# Autodesk Inventor assembly: waterjet assembly version
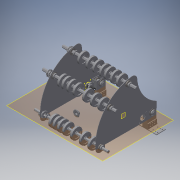
[picture p0: Inventor's stored thumbnail of the model, 180x180]
Saved by Autodesk Inventor 2018 (Build 220112000, 112)
## iProperties
Created: 2020-01-24
Part Number: waterjet assembly version
Document SubType Name: Assembly
Designer: s-2513225
Author: s-2513225
## Documents named in this file (11)
- \\studenthome\students\S-2513225\GitHub\2020CAD\Over bumper intake\Assembly\waterjet assembly version.iam
- \\studenthome\students\S-2513225\GitHub\2020CAD\Over bumper intake\Parts\waterjet wall.ipt
- \\studenthome\students\S-2513225\GitHub\2020CAD\Over bumper intake\Parts\0_500_Hex_ID_x_1_125_OD_x_0_313_WD_Flanged_Bearing_v2_217-3875.ipt
- \\studenthome\students\S-2513225\GitHub\2020CAD\Over bumper intake\Parts\hex shaft 1.ipt
- \\studenthome\students\S-2513225\GitHub\2020CAD\Over bumper intake\Parts\banebots 400 - 2 3-8 replacement.ipt
- \\studenthome\students\S-2513225\GitHub\2020CAD\Over bumper intake\Parts\anchor point.ipt
- \\studenthome\students\S-2513225\GitHub\2020CAD\Over bumper intake\Parts\hex 2.ipt
- \\studenthome\students\S-2513225\GitHub\2020CAD\Over bumper intake\Parts\2in bracket.ipt
- \\studenthome\students\S-2513225\GitHub\2020CAD\Over bumper intake\Parts\VersaPlanetary_v2_Single_Stage_10_1_with_775_Series.iam
- \\studenthome\students\S-2513225\GitHub\2020CAD\Over bumper intake\Parts\_16t_Aluminum_Hub_Sprocket_25_Chain_1_2_Hex_Bore_217-2642.ipt
- \\studenthome\students\S-2513225\GitHub\2020CAD\Over bumper intake\Parts\Clamping_Shaft_Collar_-_1_2_Hex_ID_217-2737.ipt
## Components (67 placed, 10 different names)
1. waterjet wall:1 — Mate:2, Mate:4, Mate:5, Mate:6, Mate:7, Mate:8, Mate:9, Mate:26, Mate:90, Mate:91, Mate:97, Mate:108, Mate:109, Flush:11, Flush:12, Mate:154, Mate:157, Mate:165
2. waterjet wall:2 — Mate:17, Mate:18, Mate:19, Mate:20, Mate:21, Mate:22, Mate:26, Mate:88, Mate:89, Mate:99, Flush:13, Mate:166
3. 0_500_Hex_ID_x_1_125_OD_x_0_313_WD_Flanged_Bearing_v2_217-3875:1 — Mate:5, Mate:7, Mate:10, Mate:15, Mate:150
4. 0_500_Hex_ID_x_1_125_OD_x_0_313_WD_Flanged_Bearing_v2_217-3875:2 — Mate:6, Mate:9, Mate:12, Mate:14, Mate:152
5. 0_500_Hex_ID_x_1_125_OD_x_0_313_WD_Flanged_Bearing_v2_217-3875:3 — Mate:4, Mate:8, Mate:11, Mate:13
6. 0_500_Hex_ID_x_1_125_OD_x_0_313_WD_Flanged_Bearing_v2_217-3875:4 — Mate:19, Mate:21, Mate:24
7. 0_500_Hex_ID_x_1_125_OD_x_0_313_WD_Flanged_Bearing_v2_217-3875:5 — Mate:18, Mate:20, Mate:23, Mate:25
8. 0_500_Hex_ID_x_1_125_OD_x_0_313_WD_Flanged_Bearing_v2_217-3875:6 — Mate:17, Mate:22
9. hex shaft 1:1 — Mate:12, Mate:14, Mate:23, Mate:25, Mate:37, Mate:53, Mate:68, Mate:72, Mate:73, Mate:74, Mate:75, Mate:76, Mate:77, Mate:78, Mate:104, Mate:105, Mate:106, Mate:107, Flush:11, Mate:122, Mate:123, Mate:138, Mate:139, Mate:153, Mate:161
10. hex shaft 1:2 — Mate:10, Mate:15, Mate:27, Mate:28, Mate:29, Mate:30, Mate:39, Mate:42, Mate:43, Mate:44, Mate:45, Mate:46, Mate:61, Mate:62, Mate:63, Mate:64, Mate:132, Mate:133, Mate:134, Mate:135, Mate:136, Mate:147, Mate:151, Mate:162
11. hex shaft 1:3 — Mate:11, Mate:13, Mate:24, Mate:31, Mate:32, Mate:33, Mate:34, Mate:40, Mate:47, Mate:48, Mate:49, Mate:50, Mate:51, Mate:65, Mate:66, Mate:69, Mate:70, Mate:124, Mate:125, Mate:126, Mate:127, Mate:128, Mate:129, Mate:137, Mate:148, Mate:163
12. banebots 400 - 2 3-8 replacement:1 — Mate:27, Mate:42
13. banebots 400 - 2 3-8 replacement:2 — Mate:30, Mate:43
14. banebots 400 - 2 3-8 replacement:3 — Mate:31, Mate:50
15. banebots 400 - 2 3-8 replacement:4 — Mate:29, Mate:44
16. banebots 400 - 2 3-8 replacement:5 — Mate:40, Mate:51
17. banebots 400 - 2 3-8 replacement:6 — Mate:28, Mate:46
18. banebots 400 - 2 3-8 replacement:7 — Mate:34, Mate:47
19. banebots 400 - 2 3-8 replacement:8 — Mate:32, Mate:48
20. banebots 400 - 2 3-8 replacement:9 — Mate:39, Mate:45
21. banebots 400 - 2 3-8 replacement:10 — Mate:73, Mate:78
22. banebots 400 - 2 3-8 replacement:11 — Mate:37, Mate:53
23. banebots 400 - 2 3-8 replacement:12 — Mate:75, Mate:76
24. banebots 400 - 2 3-8 replacement:13 — Mate:105, Mate:106
25. banebots 400 - 2 3-8 replacement:14 — Mate:33, Mate:49
26. banebots 400 - 2 3-8 replacement:15 — Mate:104, Mate:107
27. banebots 400 - 2 3-8 replacement:16 — Mate:61, Mate:63
28. banebots 400 - 2 3-8 replacement:17 — Mate:62, Mate:64
29. banebots 400 - 2 3-8 replacement:18 — Mate:66, Mate:70
30. banebots 400 - 2 3-8 replacement:19 — Mate:65, Mate:69
31. banebots 400 - 2 3-8 replacement:20 — Mate:74, Mate:77
32. banebots 400 - 2 3-8 replacement:21 — Mate:68, Mate:72
33. anchor point:1 — Mate:80, Mate:81, Mate:97, Flush:5, Mate:101, Flush:6, Flush:9, Flush:10, Mate:103, Mate:164, Mate:168
34. anchor point:2 — Mate:86, Mate:87, Mate:99, Mate:100, Flush:3, Flush:4, Mate:102, Flush:7, Flush:8, Mate:167
35. 0_500_Hex_ID_x_1_125_OD_x_0_313_WD_Flanged_Bearing_v2_217-3875:7 — Mate:80, Mate:81, Mate:96
36. 0_500_Hex_ID_x_1_125_OD_x_0_313_WD_Flanged_Bearing_v2_217-3875:10 — Mate:86, Mate:87
37. 0_500_Hex_ID_x_1_125_OD_x_0_313_WD_Flanged_Bearing_v2_217-3875:11 — Mate:88, Mate:89, Mate:92, Mate:94, Mate:167
38. 0_500_Hex_ID_x_1_125_OD_x_0_313_WD_Flanged_Bearing_v2_217-3875:12 — Mate:90, Mate:91, Mate:93, Mate:95, Mate:168
39. hex 2:1 — Mate:93, Mate:95, Mate:96, Mate:110, Mate:111, Mate:112, Mate:113
40. hex 2:2 — Mate:92, Mate:94, Mate:114, Mate:115, Mate:116, Mate:117
41. 2in bracket:1 — Flush:5, Mate:101, Flush:6, Flush:12
42. 2in bracket:2 — Mate:100, Flush:3, Flush:4, Flush:13
43. 2in bracket:3 — Mate:102, Flush:7, Flush:8
44. 2in bracket:4 — Flush:9, Flush:10, Mate:103
45. VersaPlanetary_v2_Single_Stage_10_1_with_775_Series:1 [sub-assembly] — Mate:144, Mate:154, Mate:157, Mate:158, Mate:159, Mate:160
46. 0_500_Hex_ID_x_1_125_OD_x_0_313_WD_Flanged_Bearing_v2_217-3875:13 — Mate:108, Mate:109, Mate:144, Mate:155
47. _16t_Aluminum_Hub_Sprocket_25_Chain_1_2_Hex_Bore_217-2642:1 — Mate:150, Mate:151
48. _16t_Aluminum_Hub_Sprocket_25_Chain_1_2_Hex_Bore_217-2642:2 — Mate:152, Mate:153, Mate:161, Mate:169, Mate:170
49. _16t_Aluminum_Hub_Sprocket_25_Chain_1_2_Hex_Bore_217-2642:4 — Mate:124, Mate:125
50. Clamping_Shaft_Collar_-_1_2_Hex_ID_217-2737:1 — Mate:122, Mate:123
51. Clamping_Shaft_Collar_-_1_2_Hex_ID_217-2737:2 — Mate:128, Mate:129
52. Clamping_Shaft_Collar_-_1_2_Hex_ID_217-2737:3 — Mate:134, Mate:135
53. Clamping_Shaft_Collar_-_1_2_Hex_ID_217-2737:4 — Mate:138, Mate:139
54. Clamping_Shaft_Collar_-_1_2_Hex_ID_217-2737:5 — Mate:137, Mate:163
55. Clamping_Shaft_Collar_-_1_2_Hex_ID_217-2737:6 — Mate:136, Mate:162
56. Clamping_Shaft_Collar_-_1_2_Hex_ID_217-2737:7 — Mate:114, Mate:115
57. Clamping_Shaft_Collar_-_1_2_Hex_ID_217-2737:8 — Mate:116, Mate:117
58. Clamping_Shaft_Collar_-_1_2_Hex_ID_217-2737:9 — Mate:110, Mate:111
59. Clamping_Shaft_Collar_-_1_2_Hex_ID_217-2737:10 — Mate:112, Mate:113
60. Clamping_Shaft_Collar_-_1_2_Hex_ID_217-2737:11 — Mate:147
61. _16t_Aluminum_Hub_Sprocket_25_Chain_1_2_Hex_Bore_217-2642:5 — Mate:126, Mate:127
62. _16t_Aluminum_Hub_Sprocket_25_Chain_1_2_Hex_Bore_217-2642:6 — Mate:132, Mate:133
63. _16t_Aluminum_Hub_Sprocket_25_Chain_1_2_Hex_Bore_217-2642:7
64. Clamping_Shaft_Collar_-_1_2_Hex_ID_217-2737:12 — Mate:159, Mate:160
65. _16t_Aluminum_Hub_Sprocket_25_Chain_1_2_Hex_Bore_217-2642:8 — Mate:155, Mate:158
66. Clamping_Shaft_Collar_-_1_2_Hex_ID_217-2737:13 — Mate:148
67. Clamping_Shaft_Collar_-_1_2_Hex_ID_217-2737:15 — Mate:169, Mate:170
## Relationships (144: Mate 133, Flush 11)
- Mate:2: waterjet wall:1
- Mate:4: waterjet wall:1 ↔ 0_500_Hex_ID_x_1_125_OD_x_0_313_WD_Flanged_Bearing_v2_217-3875:3
- Mate:5: waterjet wall:1 ↔ 0_500_Hex_ID_x_1_125_OD_x_0_313_WD_Flanged_Bearing_v2_217-3875:1
- Mate:6: waterjet wall:1 ↔ 0_500_Hex_ID_x_1_125_OD_x_0_313_WD_Flanged_Bearing_v2_217-3875:2
- Mate:7: waterjet wall:1 ↔ 0_500_Hex_ID_x_1_125_OD_x_0_313_WD_Flanged_Bearing_v2_217-3875:1
- Mate:8: waterjet wall:1 ↔ 0_500_Hex_ID_x_1_125_OD_x_0_313_WD_Flanged_Bearing_v2_217-3875:3
- Mate:9: waterjet wall:1 ↔ 0_500_Hex_ID_x_1_125_OD_x_0_313_WD_Flanged_Bearing_v2_217-3875:2
- Mate:10: 0_500_Hex_ID_x_1_125_OD_x_0_313_WD_Flanged_Bearing_v2_217-3875:1 ↔ hex shaft 1:2
- Mate:11: 0_500_Hex_ID_x_1_125_OD_x_0_313_WD_Flanged_Bearing_v2_217-3875:3 ↔ hex shaft 1:3
- Mate:12: 0_500_Hex_ID_x_1_125_OD_x_0_313_WD_Flanged_Bearing_v2_217-3875:2 ↔ hex shaft 1:1
- Mate:13: 0_500_Hex_ID_x_1_125_OD_x_0_313_WD_Flanged_Bearing_v2_217-3875:3 ↔ hex shaft 1:3
- Mate:14: 0_500_Hex_ID_x_1_125_OD_x_0_313_WD_Flanged_Bearing_v2_217-3875:2 ↔ hex shaft 1:1
- Mate:15: 0_500_Hex_ID_x_1_125_OD_x_0_313_WD_Flanged_Bearing_v2_217-3875:1 ↔ hex shaft 1:2
- Mate:17: waterjet wall:2 ↔ 0_500_Hex_ID_x_1_125_OD_x_0_313_WD_Flanged_Bearing_v2_217-3875:6
- Mate:18: waterjet wall:2 ↔ 0_500_Hex_ID_x_1_125_OD_x_0_313_WD_Flanged_Bearing_v2_217-3875:5
- Mate:19: waterjet wall:2 ↔ 0_500_Hex_ID_x_1_125_OD_x_0_313_WD_Flanged_Bearing_v2_217-3875:4
- Mate:20: waterjet wall:2 ↔ 0_500_Hex_ID_x_1_125_OD_x_0_313_WD_Flanged_Bearing_v2_217-3875:5
- Mate:21: waterjet wall:2 ↔ 0_500_Hex_ID_x_1_125_OD_x_0_313_WD_Flanged_Bearing_v2_217-3875:4
- Mate:22: waterjet wall:2 ↔ 0_500_Hex_ID_x_1_125_OD_x_0_313_WD_Flanged_Bearing_v2_217-3875:6
- Mate:23: 0_500_Hex_ID_x_1_125_OD_x_0_313_WD_Flanged_Bearing_v2_217-3875:5 ↔ hex shaft 1:1
- Mate:24: 0_500_Hex_ID_x_1_125_OD_x_0_313_WD_Flanged_Bearing_v2_217-3875:4 ↔ hex shaft 1:3
- Mate:25: 0_500_Hex_ID_x_1_125_OD_x_0_313_WD_Flanged_Bearing_v2_217-3875:5 ↔ hex shaft 1:1
- Mate:26 (304.8 mm): waterjet wall:1 ↔ waterjet wall:2
- Mate:27: hex shaft 1:2 ↔ banebots 400 - 2 3-8 replacement:1
- Mate:28: hex shaft 1:2 ↔ banebots 400 - 2 3-8 replacement:6
- Mate:29: hex shaft 1:2 ↔ banebots 400 - 2 3-8 replacement:4
- Mate:30: hex shaft 1:2 ↔ banebots 400 - 2 3-8 replacement:2
- Mate:31: hex shaft 1:3 ↔ banebots 400 - 2 3-8 replacement:3
- Mate:32: hex shaft 1:3 ↔ banebots 400 - 2 3-8 replacement:8
- Mate:33: hex shaft 1:3 ↔ banebots 400 - 2 3-8 replacement:14
- Mate:34: hex shaft 1:3 ↔ banebots 400 - 2 3-8 replacement:7
- Mate:37: hex shaft 1:1 ↔ banebots 400 - 2 3-8 replacement:11
- Mate:39: hex shaft 1:2 ↔ banebots 400 - 2 3-8 replacement:9
- Mate:40: hex shaft 1:3 ↔ banebots 400 - 2 3-8 replacement:5
- Mate:42: hex shaft 1:2 ↔ banebots 400 - 2 3-8 replacement:1
- Mate:43: hex shaft 1:2 ↔ banebots 400 - 2 3-8 replacement:2
- Mate:44: hex shaft 1:2 ↔ banebots 400 - 2 3-8 replacement:4
- Mate:45: hex shaft 1:2 ↔ banebots 400 - 2 3-8 replacement:9
- Mate:46: hex shaft 1:2 ↔ banebots 400 - 2 3-8 replacement:6
- Mate:47: hex shaft 1:3 ↔ banebots 400 - 2 3-8 replacement:7
- Mate:48: hex shaft 1:3 ↔ banebots 400 - 2 3-8 replacement:8
- Mate:49: hex shaft 1:3 ↔ banebots 400 - 2 3-8 replacement:14
- Mate:50: hex shaft 1:3 ↔ banebots 400 - 2 3-8 replacement:3
- Mate:51: hex shaft 1:3 ↔ banebots 400 - 2 3-8 replacement:5
- Mate:53: hex shaft 1:1 ↔ banebots 400 - 2 3-8 replacement:11
- Mate:61: hex shaft 1:2 ↔ banebots 400 - 2 3-8 replacement:16
- Mate:62: hex shaft 1:2 ↔ banebots 400 - 2 3-8 replacement:17
- Mate:63: hex shaft 1:2 ↔ banebots 400 - 2 3-8 replacement:16
- Mate:64: hex shaft 1:2 ↔ banebots 400 - 2 3-8 replacement:17
- Mate:65: hex shaft 1:3 ↔ banebots 400 - 2 3-8 replacement:19
- Mate:66: hex shaft 1:3 ↔ banebots 400 - 2 3-8 replacement:18
- Mate:68: hex shaft 1:1 ↔ banebots 400 - 2 3-8 replacement:21
- Mate:69: hex shaft 1:3 ↔ banebots 400 - 2 3-8 replacement:19
- Mate:70: hex shaft 1:3 ↔ banebots 400 - 2 3-8 replacement:18
- Mate:72: hex shaft 1:1 ↔ banebots 400 - 2 3-8 replacement:21
- Mate:73: hex shaft 1:1 ↔ banebots 400 - 2 3-8 replacement:10
- Mate:74: hex shaft 1:1 ↔ banebots 400 - 2 3-8 replacement:20
- Mate:75: hex shaft 1:1 ↔ banebots 400 - 2 3-8 replacement:12
- Mate:76: hex shaft 1:1 ↔ banebots 400 - 2 3-8 replacement:12
- Mate:77: hex shaft 1:1 ↔ banebots 400 - 2 3-8 replacement:20
- Mate:78: hex shaft 1:1 ↔ banebots 400 - 2 3-8 replacement:10
- Mate:80: anchor point:1 ↔ 0_500_Hex_ID_x_1_125_OD_x_0_313_WD_Flanged_Bearing_v2_217-3875:7
- Mate:81: anchor point:1 ↔ 0_500_Hex_ID_x_1_125_OD_x_0_313_WD_Flanged_Bearing_v2_217-3875:7
- Mate:86: anchor point:2 ↔ 0_500_Hex_ID_x_1_125_OD_x_0_313_WD_Flanged_Bearing_v2_217-3875:10
- Mate:87: anchor point:2 ↔ 0_500_Hex_ID_x_1_125_OD_x_0_313_WD_Flanged_Bearing_v2_217-3875:10
- Mate:88: waterjet wall:2 ↔ 0_500_Hex_ID_x_1_125_OD_x_0_313_WD_Flanged_Bearing_v2_217-3875:11
- Mate:89: waterjet wall:2 ↔ 0_500_Hex_ID_x_1_125_OD_x_0_313_WD_Flanged_Bearing_v2_217-3875:11
- Mate:90: waterjet wall:1 ↔ 0_500_Hex_ID_x_1_125_OD_x_0_313_WD_Flanged_Bearing_v2_217-3875:12
- Mate:91: waterjet wall:1 ↔ 0_500_Hex_ID_x_1_125_OD_x_0_313_WD_Flanged_Bearing_v2_217-3875:12
- Mate:92: 0_500_Hex_ID_x_1_125_OD_x_0_313_WD_Flanged_Bearing_v2_217-3875:11 ↔ hex 2:2
- Mate:93: 0_500_Hex_ID_x_1_125_OD_x_0_313_WD_Flanged_Bearing_v2_217-3875:12 ↔ hex 2:1
- Mate:94: 0_500_Hex_ID_x_1_125_OD_x_0_313_WD_Flanged_Bearing_v2_217-3875:11 ↔ hex 2:2
- Mate:95: 0_500_Hex_ID_x_1_125_OD_x_0_313_WD_Flanged_Bearing_v2_217-3875:12 ↔ hex 2:1
- Mate:96: 0_500_Hex_ID_x_1_125_OD_x_0_313_WD_Flanged_Bearing_v2_217-3875:7 ↔ hex 2:1
- Mate:97: waterjet wall:1 ↔ anchor point:1
- Mate:99: waterjet wall:2 ↔ anchor point:2
- Mate:100: anchor point:2 ↔ 2in bracket:2
- Flush:3: anchor point:2 ↔ 2in bracket:2
- Flush:4: anchor point:2 ↔ 2in bracket:2
- Flush:5: anchor point:1 ↔ 2in bracket:1
- Mate:101: anchor point:1 ↔ 2in bracket:1
- Flush:6: anchor point:1 ↔ 2in bracket:1
- Mate:102: anchor point:2 ↔ 2in bracket:3
- Flush:7: anchor point:2 ↔ 2in bracket:3
- Flush:8: anchor point:2 ↔ 2in bracket:3
- Flush:9: anchor point:1 ↔ 2in bracket:4
- Flush:10: anchor point:1 ↔ 2in bracket:4
- Mate:103: anchor point:1 ↔ 2in bracket:4
- Mate:104: hex shaft 1:1 ↔ banebots 400 - 2 3-8 replacement:15
- Mate:105: hex shaft 1:1 ↔ banebots 400 - 2 3-8 replacement:13
- Mate:106: hex shaft 1:1 ↔ banebots 400 - 2 3-8 replacement:13
- Mate:107: hex shaft 1:1 ↔ banebots 400 - 2 3-8 replacement:15
- Mate:108: waterjet wall:1 ↔ 0_500_Hex_ID_x_1_125_OD_x_0_313_WD_Flanged_Bearing_v2_217-3875:13
- Mate:109: waterjet wall:1 ↔ 0_500_Hex_ID_x_1_125_OD_x_0_313_WD_Flanged_Bearing_v2_217-3875:13
- Mate:110 (1.27 mm): hex 2:1 ↔ Clamping_Shaft_Collar_-_1_2_Hex_ID_217-2737:9
- Mate:111 (1.27 mm): hex 2:1 ↔ Clamping_Shaft_Collar_-_1_2_Hex_ID_217-2737:9
- Mate:112 (1.27 mm): hex 2:1 ↔ Clamping_Shaft_Collar_-_1_2_Hex_ID_217-2737:10
- Mate:113 (1.27 mm): hex 2:1 ↔ Clamping_Shaft_Collar_-_1_2_Hex_ID_217-2737:10
- Mate:114 (1.27 mm): hex 2:2 ↔ Clamping_Shaft_Collar_-_1_2_Hex_ID_217-2737:7
- Mate:115 (1.27 mm): hex 2:2 ↔ Clamping_Shaft_Collar_-_1_2_Hex_ID_217-2737:7
- Mate:116 (1.27 mm): hex 2:2 ↔ Clamping_Shaft_Collar_-_1_2_Hex_ID_217-2737:8
- Mate:117 (1.27 mm): hex 2:2 ↔ Clamping_Shaft_Collar_-_1_2_Hex_ID_217-2737:8
- Flush:11 (50.8 mm): waterjet wall:1 ↔ hex shaft 1:1
- Mate:122: hex shaft 1:1 ↔ Clamping_Shaft_Collar_-_1_2_Hex_ID_217-2737:1
- Mate:123 (1.27 mm): hex shaft 1:1 ↔ Clamping_Shaft_Collar_-_1_2_Hex_ID_217-2737:1
- Mate:124 (1.27 mm): hex shaft 1:3 ↔ _16t_Aluminum_Hub_Sprocket_25_Chain_1_2_Hex_Bore_217-2642:4
- Mate:125: hex shaft 1:3 ↔ _16t_Aluminum_Hub_Sprocket_25_Chain_1_2_Hex_Bore_217-2642:4
- Mate:126 (1.27 mm): hex shaft 1:3 ↔ _16t_Aluminum_Hub_Sprocket_25_Chain_1_2_Hex_Bore_217-2642:5
- Mate:127: hex shaft 1:3 ↔ _16t_Aluminum_Hub_Sprocket_25_Chain_1_2_Hex_Bore_217-2642:5
- Mate:128 (1.27 mm): hex shaft 1:3 ↔ Clamping_Shaft_Collar_-_1_2_Hex_ID_217-2737:2
- Mate:129: hex shaft 1:3 ↔ Clamping_Shaft_Collar_-_1_2_Hex_ID_217-2737:2
- Mate:132 (1.27 mm): hex shaft 1:2 ↔ _16t_Aluminum_Hub_Sprocket_25_Chain_1_2_Hex_Bore_217-2642:6
- Mate:133: hex shaft 1:2 ↔ _16t_Aluminum_Hub_Sprocket_25_Chain_1_2_Hex_Bore_217-2642:6
- Mate:134 (1.27 mm): hex shaft 1:2 ↔ Clamping_Shaft_Collar_-_1_2_Hex_ID_217-2737:3
- Mate:135: hex shaft 1:2 ↔ Clamping_Shaft_Collar_-_1_2_Hex_ID_217-2737:3
- Mate:136 (1.27 mm): hex shaft 1:2 ↔ Clamping_Shaft_Collar_-_1_2_Hex_ID_217-2737:6
- Mate:137 (1.27 mm): hex shaft 1:3 ↔ Clamping_Shaft_Collar_-_1_2_Hex_ID_217-2737:5
- Mate:138 (1.27 mm): hex shaft 1:1 ↔ Clamping_Shaft_Collar_-_1_2_Hex_ID_217-2737:4
- Mate:139: hex shaft 1:1 ↔ Clamping_Shaft_Collar_-_1_2_Hex_ID_217-2737:4
- Mate:144: VersaPlanetary_v2_Single_Stage_10_1_with_775_Series:1 ↔ 0_500_Hex_ID_x_1_125_OD_x_0_313_WD_Flanged_Bearing_v2_217-3875:13
- Flush:12 (-48.768 mm): waterjet wall:1 ↔ 2in bracket:1
- Flush:13 (-48.768 mm): waterjet wall:2 ↔ 2in bracket:2
- Mate:147 (1.27 mm): hex shaft 1:2 ↔ Clamping_Shaft_Collar_-_1_2_Hex_ID_217-2737:11
- Mate:148 (1.27 mm): hex shaft 1:3 ↔ Clamping_Shaft_Collar_-_1_2_Hex_ID_217-2737:13
- Mate:150: 0_500_Hex_ID_x_1_125_OD_x_0_313_WD_Flanged_Bearing_v2_217-3875:1 ↔ _16t_Aluminum_Hub_Sprocket_25_Chain_1_2_Hex_Bore_217-2642:1
- Mate:151 (1.27 mm): hex shaft 1:2 ↔ _16t_Aluminum_Hub_Sprocket_25_Chain_1_2_Hex_Bore_217-2642:1
- Mate:152: 0_500_Hex_ID_x_1_125_OD_x_0_313_WD_Flanged_Bearing_v2_217-3875:2 ↔ _16t_Aluminum_Hub_Sprocket_25_Chain_1_2_Hex_Bore_217-2642:2
- Mate:153 (1.27 mm): hex shaft 1:1 ↔ _16t_Aluminum_Hub_Sprocket_25_Chain_1_2_Hex_Bore_217-2642:2
- Mate:154: waterjet wall:1 ↔ VersaPlanetary_v2_Single_Stage_10_1_with_775_Series:1
- Mate:155: 0_500_Hex_ID_x_1_125_OD_x_0_313_WD_Flanged_Bearing_v2_217-3875:13 ↔ _16t_Aluminum_Hub_Sprocket_25_Chain_1_2_Hex_Bore_217-2642:8
- Mate:157: waterjet wall:1 ↔ VersaPlanetary_v2_Single_Stage_10_1_with_775_Series:1
- Mate:158: VersaPlanetary_v2_Single_Stage_10_1_with_775_Series:1 ↔ _16t_Aluminum_Hub_Sprocket_25_Chain_1_2_Hex_Bore_217-2642:8
- Mate:159: VersaPlanetary_v2_Single_Stage_10_1_with_775_Series:1 ↔ Clamping_Shaft_Collar_-_1_2_Hex_ID_217-2737:12
- Mate:160: VersaPlanetary_v2_Single_Stage_10_1_with_775_Series:1 ↔ Clamping_Shaft_Collar_-_1_2_Hex_ID_217-2737:12
- Mate:161: hex shaft 1:1 ↔ _16t_Aluminum_Hub_Sprocket_25_Chain_1_2_Hex_Bore_217-2642:2
- Mate:162 (1.27 mm): hex shaft 1:2 ↔ Clamping_Shaft_Collar_-_1_2_Hex_ID_217-2737:6
- Mate:163 (1.27 mm): hex shaft 1:3 ↔ Clamping_Shaft_Collar_-_1_2_Hex_ID_217-2737:5
- Mate:164: anchor point:1
- Mate:165: waterjet wall:1
- Mate:166: waterjet wall:2
- Mate:167: anchor point:2 ↔ 0_500_Hex_ID_x_1_125_OD_x_0_313_WD_Flanged_Bearing_v2_217-3875:11
- Mate:168: anchor point:1 ↔ 0_500_Hex_ID_x_1_125_OD_x_0_313_WD_Flanged_Bearing_v2_217-3875:12
- Mate:169: _16t_Aluminum_Hub_Sprocket_25_Chain_1_2_Hex_Bore_217-2642:2 ↔ Clamping_Shaft_Collar_-_1_2_Hex_ID_217-2737:15
- Mate:170: _16t_Aluminum_Hub_Sprocket_25_Chain_1_2_Hex_Bore_217-2642:2 ↔ Clamping_Shaft_Collar_-_1_2_Hex_ID_217-2737:15
